# Autodesk Inventor assembly: Doboz
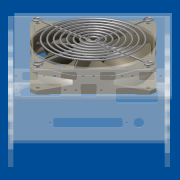
[picture p0: Inventor's stored thumbnail of the model, 180x180]
Saved by Autodesk Inventor 2015 SP1 (Build 190203100, 203)
## iProperties
Created: 2013-02-23
Part Number: Doboz
Document SubType Name: Weldment
Designer: laca
Weld Material: Default
Author: laca
## Documents named in this file (10)
- G:\egyetemMent\iRoobo2013\AlaplapDoboz\Doboz.iam
- G:\egyetemMent\iRoobo2013\AlaplapDoboz\NagyLap2.ipt
- G:\egyetemMent\iRoobo2013\AlaplapDoboz\ventilatorIn.ipt
- G:\egyetemMent\iRoobo2013\AlaplapDoboz\PC Fan grill.ipt
- G:\egyetemMent\iRoobo2013\AlaplapDoboz\OldalalKicsi1.ipt
- G:\egyetemMent\iRoobo2013\AlaplapDoboz\OldalapNagy1.ipt
- G:\egyetemMent\iRoobo2013\AlaplapDoboz\NagyLap1.ipt
- G:\egyetemMent\iRoobo2013\AlaplapDoboz\Elolap.ipt
- G:\egyetemMent\iRoobo2013\AlaplapDoboz\Sarok.ipt
- G:\egyetemMent\iRoobo2013\ForgoSarok.iam
## Components (11 placed, 9 different names)
1. NagyLap2:1 — Mate:1, Mate:2, Mate:3, Insert:1, Insert:2, Mate:12, Flush:1, Mate:24, Mate:28, Mate:29
2. ventilatorIn:1 — Insert:1, Insert:2
3. PC Fan grill:1 — Mate:1, Mate:2, Mate:3
4. OldalalKicsi1:1 — Mate:12, Flush:1, Flush:4, Mate:17, Mate:23, Flush:7, Mate:27, Flush:8, Mate:31, Flush:9, Mate:32, Flush:10, Mate:36, Mate:37, Tangent:2
5. OldalapNagy1:1 — Flush:4, Mate:17, Mate:23, Mate:24, Flush:7, Mate:33, Mate:38
6. NagyLap1:1 — Mate:34, Flush:11, Flush:12, Mate:35, Tangent:1, Flush:13
7. Elolap:1 — Mate:34, Flush:11, Flush:12, Mate:38
8. Sarok:1 — Mate:32, Mate:33, Flush:10
9. Sarok:2 — Mate:30, Mate:31, Flush:9
10. OldalapNagy1:2 — Mate:27, Flush:8, Mate:28, Mate:29, Mate:30
11. ForgoSarok:1 [sub-assembly] — Mate:35, Tangent:1, Flush:13, Mate:36, Mate:37, Tangent:2
## Relationships (32: Mate 19, Flush 9, Insert 2, Tangent 2)
- Mate:1: NagyLap2:1 ↔ PC Fan grill:1
- Mate:2 (2 mm): NagyLap2:1 ↔ PC Fan grill:1
- Mate:3: NagyLap2:1 ↔ PC Fan grill:1
- Insert:1: NagyLap2:1 ↔ ventilatorIn:1
- Insert:2: NagyLap2:1 ↔ ventilatorIn:1
- Mate:12: NagyLap2:1 ↔ OldalalKicsi1:1
- Flush:1: NagyLap2:1 ↔ OldalalKicsi1:1
- Flush:4: OldalalKicsi1:1 ↔ OldalapNagy1:1
- Mate:17: OldalalKicsi1:1 ↔ OldalapNagy1:1
- Mate:23: OldalalKicsi1:1 ↔ OldalapNagy1:1
- Mate:24: NagyLap2:1 ↔ OldalapNagy1:1
- Flush:7: OldalalKicsi1:1 ↔ OldalapNagy1:1
- Mate:27: OldalalKicsi1:1 ↔ OldalapNagy1:2
- Flush:8: OldalalKicsi1:1 ↔ OldalapNagy1:2
- Mate:28: NagyLap2:1 ↔ OldalapNagy1:2
- Mate:29 (2 mm): NagyLap2:1 ↔ OldalapNagy1:2
- Mate:30: Sarok:2 ↔ OldalapNagy1:2
- Mate:31: OldalalKicsi1:1 ↔ Sarok:2
- Flush:9: OldalalKicsi1:1 ↔ Sarok:2
- Mate:32: OldalalKicsi1:1 ↔ Sarok:1
- Mate:33: OldalapNagy1:1 ↔ Sarok:1
- Flush:10: OldalalKicsi1:1 ↔ Sarok:1
- Mate:34: NagyLap1:1 ↔ Elolap:1
- Flush:11 (2 mm): NagyLap1:1 ↔ Elolap:1
- Flush:12: NagyLap1:1 ↔ Elolap:1
- Mate:35: NagyLap1:1 ↔ ForgoSarok:1
- Tangent:1: NagyLap1:1 ↔ ForgoSarok:1
- Flush:13 (60 mm): NagyLap1:1 ↔ ForgoSarok:1
- Mate:36: OldalalKicsi1:1 ↔ ForgoSarok:1
- Mate:37: OldalalKicsi1:1 ↔ ForgoSarok:1
- Mate:38 (-1.5 mm): OldalapNagy1:1 ↔ Elolap:1
- Tangent:2 (-1 mm): OldalalKicsi1:1 ↔ ForgoSarok:1
